# Autodesk Inventor assembly: VerticalElectronicsBar
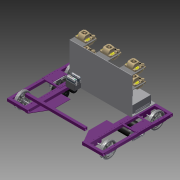
[picture p0: Inventor's stored thumbnail of the model, 180x180]
Saved by Autodesk Inventor 2012 (Build 160160000, 160)
## iProperties
Created: 2012-01-10
Part Number: VerticalElectronicsBar
Document SubType Name: Assembly
Designer: William
Author: William
## Documents named in this file (11)
- C:\Users\William\Dropbox\Robotics\CAD\team1885frc\Robot2012\Concepts\Electronics Board\VerticalElectronicsBarAlternativePowerSupplyMounting.iam
- C:\Users\William\Dropbox\Robotics\CAD\team1885frc\Robot2012\DriveTrain\DiveTrain_FullAssembly.iam
- C:\Users\William\Dropbox\Robotics\CAD\team1885frc\Robot2012\Concepts\Electronics Board\24in-by-14in_electronics_board.ipt
- C:\Users\William\Dropbox\Robotics\CAD\team1885frc\Robot2012\Concepts\Electronics Board\ElectronicsBoardVerticalBottom.ipt
- C:\Users\William\Dropbox\Robotics\CAD\team1885frc\Robot2012\Concepts\Electronics Board\BatteryInMount.iam
- C:\Users\William\Dropbox\Robotics\CAD\team1885frc\Electronics\cRIO_7Slot\NI Controller.iam
- C:\Users\William\Dropbox\Robotics\CAD\team1885frc\Robot2012\Concepts\Electronics Board\DualJagSettup.iam
- C:\Users\William\Dropbox\Robotics\CAD\team1885frc\Electronics\PowerDistributionBoard\elc_Power_Distro_inv.iam
- C:\Users\William\Dropbox\Robotics\CAD\team1885frc\Electronics\DigitalSidecar\elc_Digital_Sidecar_inv.iam
- C:\Users\William\Dropbox\Robotics\CAD\team1885frc\Electronics\Breaker\Breaker.iam
- C:\Users\William\Dropbox\Robotics\CAD\team1885frc\Electronics\Spike\Spike.iam
## Components (15 placed, 10 different names)
1. DiveTrain_FullAssembly:1 [sub-assembly] — Mate:1, Flush:1, Mate:3, Mate:5
2. 24in-by-14in_electronics_board:1 — Mate:1, Flush:1, Mate:3, Flush:2, Mate:4, Mate:10, Mate:11, Mate:12, Mate:13, Mate:14, Flush:5, Flush:6, Flush:7, Flush:8, Flush:9, Flush:11, Flush:12, Mate:28, Mate:32
3. ElectronicsBoardVerticalBottom:1 — Flush:2, Mate:4, Mate:5, Mate:6, Flush:3, Flush:4, Mate:7, Mate:21, Flush:14, Mate:22, Angle:3, Mate:24, Mate:25, Mate:30, Mate:31
4. BatteryInMount:1 [sub-assembly] — Mate:6, Flush:3, Flush:4
5. NI Controller:1 [sub-assembly] — Mate:7, Flush:14, Mate:22, Mate:23
6. DualJagSettup:1 [sub-assembly] — Mate:10, Flush:12, Mate:17
7. DualJagSettup:2 [sub-assembly] — Mate:11, Flush:9, Mate:16
8. DualJagSettup:3 [sub-assembly] — Mate:12, Flush:7, Flush:8, Mate:16, Mate:17
9. DualJagSettup:4 [sub-assembly] — Mate:13, Flush:11, Mate:15, Mate:29
10. DualJagSettup:5 [sub-assembly] — Mate:14, Flush:5, Flush:6, Mate:15
11. elc_Power_Distro_inv:1 [sub-assembly] — Mate:28, Mate:29
12. elc_Digital_Sidecar_inv:1 [sub-assembly] — Mate:21, Angle:3, Mate:23, Mate:24
13. Breaker:2 [sub-assembly] — Mate:25
14. Spike:1 [sub-assembly] — Mate:30, Mate:33, Flush:15
15. Spike:2 [sub-assembly] — Mate:31, Mate:32, Mate:33, Flush:15
## Relationships (39: Mate 25, Flush 13, Angle 1)
- Mate:1: DiveTrain_FullAssembly:1 ↔ 24in-by-14in_electronics_board:1
- Flush:1 (12.7 mm): DiveTrain_FullAssembly:1 ↔ 24in-by-14in_electronics_board:1
- Mate:3 (44.45 mm): DiveTrain_FullAssembly:1 ↔ 24in-by-14in_electronics_board:1
- Flush:2: 24in-by-14in_electronics_board:1 ↔ ElectronicsBoardVerticalBottom:1
- Mate:4: 24in-by-14in_electronics_board:1 ↔ ElectronicsBoardVerticalBottom:1
- Mate:5: DiveTrain_FullAssembly:1 ↔ ElectronicsBoardVerticalBottom:1
- Mate:6: ElectronicsBoardVerticalBottom:1 ↔ BatteryInMount:1
- Flush:3 (22.479 mm): ElectronicsBoardVerticalBottom:1 ↔ BatteryInMount:1
- Flush:4 (-6.35 mm): ElectronicsBoardVerticalBottom:1 ↔ BatteryInMount:1
- Mate:7: ElectronicsBoardVerticalBottom:1 ↔ NI Controller:1
- Mate:10: 24in-by-14in_electronics_board:1 ↔ DualJagSettup:1
- Mate:11: 24in-by-14in_electronics_board:1 ↔ DualJagSettup:2
- Mate:12: 24in-by-14in_electronics_board:1 ↔ DualJagSettup:3
- Mate:13: 24in-by-14in_electronics_board:1 ↔ DualJagSettup:4
- Mate:14: 24in-by-14in_electronics_board:1 ↔ DualJagSettup:5
- Flush:5: 24in-by-14in_electronics_board:1 ↔ DualJagSettup:5
- Flush:6: 24in-by-14in_electronics_board:1 ↔ DualJagSettup:5
- Flush:7: 24in-by-14in_electronics_board:1 ↔ DualJagSettup:3
- Flush:8: 24in-by-14in_electronics_board:1 ↔ DualJagSettup:3
- Flush:9: 24in-by-14in_electronics_board:1 ↔ DualJagSettup:2
- Flush:11: 24in-by-14in_electronics_board:1 ↔ DualJagSettup:4
- Mate:15 (20.32 mm): DualJagSettup:4 ↔ DualJagSettup:5
- Mate:16 (20.32 mm): DualJagSettup:2 ↔ DualJagSettup:3
- Flush:12: 24in-by-14in_electronics_board:1 ↔ DualJagSettup:1
- Mate:17 (114.3 mm): DualJagSettup:1 ↔ DualJagSettup:3
- Mate:21: ElectronicsBoardVerticalBottom:1 ↔ elc_Digital_Sidecar_inv:1
- Flush:14 (12.7 mm): ElectronicsBoardVerticalBottom:1 ↔ NI Controller:1
- Mate:22 (-25.4 mm): ElectronicsBoardVerticalBottom:1 ↔ NI Controller:1
- Angle:3 (180 deg): ElectronicsBoardVerticalBottom:1 ↔ elc_Digital_Sidecar_inv:1
- Mate:23 (25.4 mm): NI Controller:1 ↔ elc_Digital_Sidecar_inv:1
- Mate:24 (-50.8 mm): ElectronicsBoardVerticalBottom:1 ↔ elc_Digital_Sidecar_inv:1
- Mate:25: ElectronicsBoardVerticalBottom:1 ↔ Breaker:2
- Mate:28: 24in-by-14in_electronics_board:1 ↔ elc_Power_Distro_inv:1
- Mate:29: DualJagSettup:4 ↔ elc_Power_Distro_inv:1
- Mate:30: ElectronicsBoardVerticalBottom:1 ↔ Spike:1
- Mate:31: ElectronicsBoardVerticalBottom:1 ↔ Spike:2
- Mate:32 (63.5 mm): 24in-by-14in_electronics_board:1 ↔ Spike:2
- Mate:33 (6.35 mm): Spike:1 ↔ Spike:2
- Flush:15: Spike:1 ↔ Spike:2
